# Autodesk Inventor assembly: Solinoid Valve Assembly
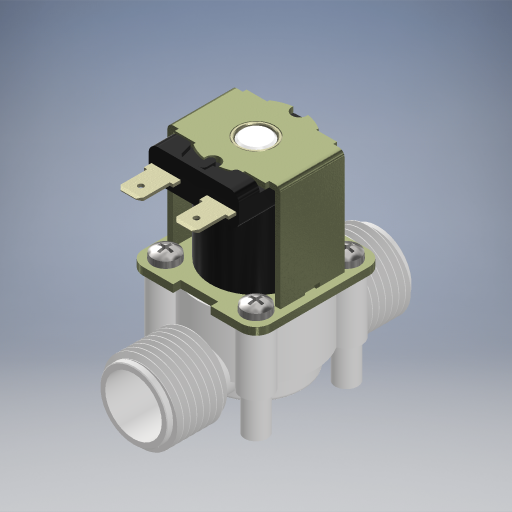
[picture p0: Inventor's stored thumbnail of the model, 512x512]
Saved by Autodesk Inventor 2024.1 (Build 281209000, 209)
## iProperties
Created: 2023-11-09
Part Number: Solinoid Valve Assembly
Document SubType Name: Assembly
Designer: Glen Collingwood
Author: Glen Collingwood
## Documents named in this file (9)
- D:\MISCELLANEOUS\Inventor Projects\Miscellaneous\Coffee Machine Mods\Solenoide Valve\Solinoid Valve Assembly.iam
- D:\MISCELLANEOUS\Inventor Projects\Miscellaneous\Coffee Machine Mods\Solenoide Valve\Body.ipt
- D:\MISCELLANEOUS\Inventor Projects\Miscellaneous\Coffee Machine Mods\Solenoide Valve\Diaphram.ipt
- D:\MISCELLANEOUS\Inventor Projects\Miscellaneous\Coffee Machine Mods\Solenoide Valve\Pressure Plate.ipt
- D:\MISCELLANEOUS\Inventor Projects\Miscellaneous\Coffee Machine Mods\Solenoide Valve\Piston.ipt
- D:\MISCELLANEOUS\Inventor Projects\Miscellaneous\Coffee Machine Mods\Solenoide Valve\Plunger.ipt
- D:\MISCELLANEOUS\Inventor Projects\Miscellaneous\Coffee Machine Mods\Solenoide Valve\Frame.ipt
- C:\Users\Glen Collingwood\Documents\Inventor\Content Center Files\R2024\en-US\ANSI B18.6.5M(16)\ANSI B18.6.5M - 3.5x1.3 x 13(9).ipt
- D:\MISCELLANEOUS\Inventor Projects\Miscellaneous\Coffee Machine Mods\Solenoide Valve\Solenoid.ipt
## Components (11 placed, 8 different names)
1. Body:1 — Mate:4, Mate:5, Mate:6, Mate:7, Flush:1, Mate:10, Mate:11, Mate:12, Flush:3
2. Pressure Plate:1 — Mate:1, Mate:2, Mate:3, Mate:5, Mate:9
3. Diaphram:1 — Mate:1, Mate:2, Mate:3, Mate:4, Mate:6
4. Piston:1 — Mate:7, Flush:1, Mate:8, Mate:13
5. Plunger:1 — Mate:8, Mate:9
6. Frame:1 — Mate:10, Mate:11, Mate:12, Insert:1, Insert:2, Insert:3, Insert:4, Flush:2
7. Cross Recessed Pan Head Tapping Screw - Type B - Type I - Metric 3.5 x 1.3 x 13:1 — Insert:1
8. Cross Recessed Pan Head Tapping Screw - Type B - Type I - Metric 3.5 x 1.3 x 13:2 — Insert:4
9. Cross Recessed Pan Head Tapping Screw - Type B - Type I - Metric 3.5 x 1.3 x 13:3 — Insert:3
10. Cross Recessed Pan Head Tapping Screw - Type B - Type I - Metric 3.5 x 1.3 x 13:4 — Insert:2
11. Solenoid:1 — Mate:13, Flush:2, Flush:3
## Relationships (20: Mate 13, Insert 4, Flush 3)
- Mate:1: Pressure Plate:1 ↔ Diaphram:1
- Mate:2: Pressure Plate:1 ↔ Diaphram:1
- Mate:3: Pressure Plate:1 ↔ Diaphram:1
- Mate:4: Body:1 ↔ Diaphram:1
- Mate:5: Body:1 ↔ Pressure Plate:1
- Mate:6: Body:1 ↔ Diaphram:1
- Mate:7: Body:1 ↔ Piston:1
- Flush:1: Body:1 ↔ Piston:1
- Mate:8: Piston:1 ↔ Plunger:1
- Mate:9: Pressure Plate:1 ↔ Plunger:1
- Mate:10: Body:1 ↔ Frame:1
- Mate:11: Body:1 ↔ Frame:1
- Mate:12: Body:1 ↔ Frame:1
- Insert:1: Frame:1 ↔ Cross Recessed Pan Head Tapping Screw - Type B - Type I - Metric 3.5 x 1.3 x 13:1
- Insert:2: Frame:1 ↔ Cross Recessed Pan Head Tapping Screw - Type B - Type I - Metric 3.5 x 1.3 x 13:4
- Insert:3: Frame:1 ↔ Cross Recessed Pan Head Tapping Screw - Type B - Type I - Metric 3.5 x 1.3 x 13:3
- Insert:4: Frame:1 ↔ Cross Recessed Pan Head Tapping Screw - Type B - Type I - Metric 3.5 x 1.3 x 13:2
- Mate:13: Piston:1 ↔ Solenoid:1
- Flush:2: Frame:1 ↔ Solenoid:1
- Flush:3: Body:1 ↔ Solenoid:1
